# Autodesk Inventor assembly: WW_10_40
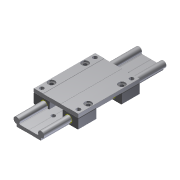
[picture p0: Inventor's stored thumbnail of the model, 180x180]
Saved by Autodesk Inventor 2014 (Build 180170000, 170)
## iProperties
Category: Miscellaneous
Company: Autodesk Inc.
Created: 2013-12-30
Part Number: WW_10_40
Document SubType Name: Assembly
Designer: Autodesk Inc.
Catalog Web Link: http://www.igus.com/wpck/3624/DryLin_W_Doppelschiene
Vendor: IGUS
Author: Autodesk Inc.
## Documents named in this file (3)
- D:\Data Folder\FIRST 2014\KOP Parts\Miscellaneous\MISC_GuideSystem_WW_10_40.iam
- D:\Data Folder\FIRST 2014\KOP Parts\Miscellaneous\MISC_Guide_WS_10_40.ipt
- D:\Data Folder\FIRST 2014\KOP Parts\Miscellaneous\MISC_GuideSystem_WW_10_40.ipt
## Components (2 placed, 2 different names)
1. MISC_Guide_WS_10_40:1 — Mate:1, Mate:2
2. MISC_GuideSystem_WW_10_40:1 — Mate:1, Mate:2
## Relationships (2: Mate 2)
- Mate:1: MISC_Guide_WS_10_40:1 ↔ MISC_GuideSystem_WW_10_40:1
- Mate:2: MISC_Guide_WS_10_40:1 ↔ MISC_GuideSystem_WW_10_40:1
